# Autodesk Inventor assembly: leg_1
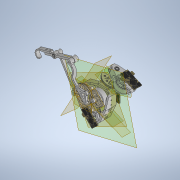
[picture p0: Inventor's stored thumbnail of the model, 180x180]
Saved by Autodesk Inventor 2020 (Build 240168000, 168)
## iProperties
Created: 2020-12-08
Part Number: leg_1
Document SubType Name: Assembly
Designer: Shuang Peng
Author: Shuang Peng
## Documents named in this file (12)
- D:\projects-3\biped_tiny\hardware\leg_1.iam
- D:\projects-3\biped_tiny\hardware\reducer_1.iam
- D:\projects-3\biped_tiny\hardware\leg_holder_2.ipt
- D:\projects-3\biped_tiny\hardware\leg_link_1.ipt
- D:\projects-3\biped_tiny\hardware\leg_link_2.ipt
- D:\projects-3\biped_tiny\hardware\leg_link_4.ipt
- D:\projects-3\biped_tiny\hardware\leg_link_3_m.ipt
- D:\projects-3\biped_tiny\hardware\foot_2.ipt
- D:\projects-3\biped_tiny\hardware\bearing_3_6_2.ipt
- D:\projects-3\biped_tiny\hardware\pin_3_15.ipt
- D:\projects-3\biped_tiny\hardware\wh_ass_3.iam
- D:\projects-3\biped_tiny\hardware\body_conn_1.ipt
## Components (22 placed, 11 different names)
1. reducer_1:1 [sub-assembly] — Flush:1, Tangent:1, Mate:4, Insert:1, Insert:2, Symmetry:1, Insert:29
2. reducer_1:2 [sub-assembly] — Flush:1, Tangent:1, Mate:3, Flush:4, Insert:3, Insert:4, Symmetry:1, Insert:30
3. leg_holder_2:1 — Flush:4, Insert:1, Insert:2, Insert:3, Insert:4, Insert:40, Insert:41, Angle:1
4. leg_link_1:1 — Flush:5, Flush:6, Insert:9, Insert:16, Flush:7, Insert:18, Insert:19, Insert:22, Insert:23, Insert:24, Insert:25
5. leg_link_2:1 — Flush:6, Insert:9, Insert:26, Insert:33, Insert:34
6. leg_link_4:1 — Insert:17, Insert:20, Insert:21, Insert:31, Insert:32
7. leg_link_3_m:1 — Insert:16, Insert:17, Insert:27, Insert:28
8. foot_2:1 — Flush:7, Insert:18, Insert:19
9. bearing_3_6_2:1 — Insert:20
10. bearing_3_6_2:2 — Insert:21
11. bearing_3_6_2:3 — Insert:23
12. bearing_3_6_2:4 — Insert:22
13. bearing_3_6_2:5 — Insert:25
14. bearing_3_6_2:6 — Insert:24
15. pin_3_15:1 — Insert:26
16. pin_3_15:2 — Insert:27
17. pin_3_15:3 — Insert:28
18. reducer_1:3 [sub-assembly] — Insert:35, Angle:1
19. wh_ass_3:1 [sub-assembly] — Insert:30, Insert:33, Insert:34
20. wh_ass_3:2 [sub-assembly] — Insert:29, Insert:31, Insert:32
21. wh_ass_3:3 [sub-assembly] — Insert:35, Insert:38, Insert:39
22. body_conn_1:1 — Insert:38, Insert:39, Insert:40, Insert:41
## Relationships (39: Insert 29, Flush 5, Mate 2, Tangent 1, Symmetry 1, Angle 1)
- Flush:1 (-9.5 mm): reducer_1:1 ↔ reducer_1:2
- Tangent:1 (2 mm): reducer_1:1 ↔ reducer_1:2
- Mate:3: reducer_1:2
- Mate:4: reducer_1:1
- Flush:4: reducer_1:2 ↔ leg_holder_2:1
- Insert:1: reducer_1:1 ↔ leg_holder_2:1
- Insert:2: reducer_1:1 ↔ leg_holder_2:1
- Insert:3: reducer_1:2 ↔ leg_holder_2:1
- Insert:4: reducer_1:2 ↔ leg_holder_2:1
- Symmetry:1: reducer_1:1 ↔ reducer_1:2
- Flush:5: leg_link_1:1
- Flush:6: leg_link_1:1 ↔ leg_link_2:1
- Insert:9: leg_link_1:1 ↔ leg_link_2:1
- Insert:16: leg_link_1:1 ↔ leg_link_3_m:1
- Insert:17: leg_link_4:1 ↔ leg_link_3_m:1
- Flush:7: leg_link_1:1 ↔ foot_2:1
- Insert:18: leg_link_1:1 ↔ foot_2:1
- Insert:19: leg_link_1:1 ↔ foot_2:1
- Insert:20: leg_link_4:1 ↔ bearing_3_6_2:1
- Insert:21: leg_link_4:1 ↔ bearing_3_6_2:2
- Insert:22: leg_link_1:1 ↔ bearing_3_6_2:4
- Insert:23: leg_link_1:1 ↔ bearing_3_6_2:3
- Insert:24: leg_link_1:1 ↔ bearing_3_6_2:6
- Insert:25: leg_link_1:1 ↔ bearing_3_6_2:5
- Insert:26: leg_link_2:1 ↔ pin_3_15:1
- Insert:27: leg_link_3_m:1 ↔ pin_3_15:2
- Insert:28: leg_link_3_m:1 ↔ pin_3_15:3
- Insert:29: reducer_1:1 ↔ wh_ass_3:2
- Insert:30: reducer_1:2 ↔ wh_ass_3:1
- Insert:31: leg_link_4:1 ↔ wh_ass_3:2
- Insert:32: leg_link_4:1 ↔ wh_ass_3:2
- Insert:33: leg_link_2:1 ↔ wh_ass_3:1
- Insert:34: leg_link_2:1 ↔ wh_ass_3:1
- Insert:35: reducer_1:3 ↔ wh_ass_3:3
- Insert:38: wh_ass_3:3 ↔ body_conn_1:1
- Insert:39: wh_ass_3:3 ↔ body_conn_1:1
- Insert:40: leg_holder_2:1 ↔ body_conn_1:1
- Insert:41: leg_holder_2:1 ↔ body_conn_1:1
- Angle:1 (0 deg): leg_holder_2:1 ↔ reducer_1:3
